# Autodesk Inventor assembly: Assembly_Cube_Eyepiece_v3
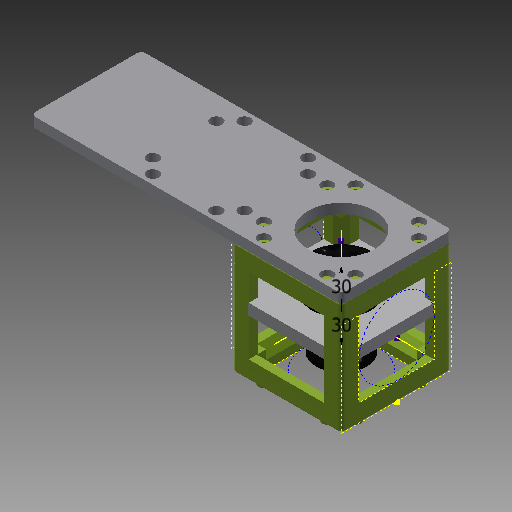
[picture p0: Inventor's stored thumbnail of the model, 512x512]
Saved by Autodesk Inventor 2019 (Build 230136000, 136)
## iProperties
Created: 2019-07-24
Part Number: Assembly_Cube_Eyepiece_v3
Document SubType Name: Assembly
Designer: marsikovabarbora
Author: marsikovabarbora
## Documents named in this file (5)
- C:\Users\marsikovabarbora\Dropbox\UC2\02_CAD\INVENTOR\uc2_v3\Assembly_Cube_Eyepiece_v3.iam
- C:\Users\marsikovabarbora\Dropbox\UC2\02_CAD\INVENTOR\uc2_v3\Assembly_Cube_empty_IM_v3.iam
- C:\Users\marsikovabarbora\Dropbox\UC2\02_CAD\INVENTOR\uc2_v3\00_Eyepiece_WF20x 23,2mm.ipt
- C:\Users\marsikovabarbora\Dropbox\UC2\02_CAD\INVENTOR\uc2_v3\30_Smartphone_Holder_v3.ipt
- C:\Users\marsikovabarbora\Dropbox\UC2\02_CAD\INVENTOR\uc2_v3\Imported Components\20_Insert_Eyepiece_v3\20_Insert_Eyepiece_v3.ipt
## Components (4 placed, 4 different names)
1. Assembly_Cube_empty_IM_v3:1 [sub-assembly] — Mate:3, Mate:4, Angle:1, Passend:5, Passend:8
2. 00_Eyepiece_WF20x 23,2mm:1 — Passend:6, Passend:7
3. 30_Smartphone_Holder_v3:1 — Mate:3, Mate:4, Angle:1
4. 20_Insert_Eyepiece_v3:1 — Passend:5, Passend:6, Passend:7, Passend:8
## Relationships (7: Mate 6, Angle 1)
- Mate:3: Assembly_Cube_empty_IM_v3:1 ↔ 30_Smartphone_Holder_v3:1
- Mate:4: Assembly_Cube_empty_IM_v3:1 ↔ 30_Smartphone_Holder_v3:1
- Angle:1 (0 deg): Assembly_Cube_empty_IM_v3:1 ↔ 30_Smartphone_Holder_v3:1
- Passend:5 [Mate]: Assembly_Cube_empty_IM_v3:1 ↔ 20_Insert_Eyepiece_v3:1
- Passend:6 [Mate]: 00_Eyepiece_WF20x 23,2mm:1 ↔ 20_Insert_Eyepiece_v3:1
- Passend:7 [Mate]: 00_Eyepiece_WF20x 23,2mm:1 ↔ 20_Insert_Eyepiece_v3:1
- Passend:8 [Mate]: Assembly_Cube_empty_IM_v3:1 ↔ 20_Insert_Eyepiece_v3:1
